# Autodesk Inventor assembly: Injector Assembly
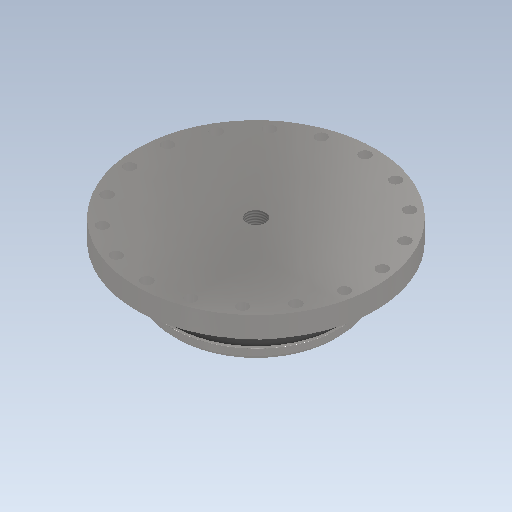
[picture p0: Inventor's stored thumbnail of the model, 512x512]
Saved by Autodesk Inventor 2021 (Build 250183000, 183)
## iProperties
Created: 2021-10-02
Part Number: Injector Assembly
Document SubType Name: Assembly
Designer: robin
Mass: 2402.63 g
Surface Area: 1092.65 cm^2
Volume: 384.578 cm^3
Density: 6.24745 g/cm^3
Author: robin
## Documents named in this file (9)
- C:\Users\alexc\OneDrive\Desktop\ATLAS\ODSY-0003 (COMBUSTION CHAMBER)\ODSY-0003-200 (INJECTOR)\ODSY-0003-200.iam
- C:\Users\alexc\OneDrive\Desktop\ATLAS\ODSY-0003 (COMBUSTION CHAMBER)\ODSY-0003-200 (INJECTOR)\ODSY-0003-201.ipt
- C:\Users\alexc\OneDrive\Desktop\ATLAS\ODSY-0003 (COMBUSTION CHAMBER)\ODSY-0003-200 (INJECTOR)\ODSY-0003-203.ipt
- C:\Users\alexc\OneDrive\Desktop\ATLAS\ODSY-0003 (COMBUSTION CHAMBER)\ODSY-0003-200 (INJECTOR)\ODSY-0003-202.ipt
- C:\Users\alexc\OneDrive\Desktop\ATLAS\ODSY-0003 (COMBUSTION CHAMBER)\ODSY-0003-200 (INJECTOR)\92185A336.ipt
- C:\Users\alexc\OneDrive\Desktop\ATLAS\ODSY-0003 (COMBUSTION CHAMBER)\ODSY-0003-200 (INJECTOR)\90945A760.ipt
- C:\Users\alexc\OneDrive\Desktop\ATLAS\ODSY-0003 (COMBUSTION CHAMBER)\ODSY-0003-200 (INJECTOR)\2-023.ipt
- C:\Users\alexc\OneDrive\Desktop\ATLAS\ODSY-0003 (COMBUSTION CHAMBER)\ODSY-0003-200 (INJECTOR)\2-030.ipt
- C:\Users\alexc\OneDrive\Desktop\ATLAS\ODSY-0003 (COMBUSTION CHAMBER)\ODSY-0003-200 (INJECTOR)\2-240.ipt
## Components (19 placed, 8 different names)
1. ODSY-0003-201:1 — Flush:1, Flush:2, Flush:3, Mate:7, Mate:8, Mate:9, Mate:10, Mate:41, Mate:42, Flush:4, Flush:5
2. ODSY-0003-203:1 — Mate:7, Mate:11, Mate:12, Mate:13, Mate:14, Mate:15, Mate:16, Mate:17, Mate:18, Mate:21, Mate:24, Mate:27, Mate:30, Mate:33, Mate:36
3. ODSY-0003-202:1 — Mate:8, Mate:9, Mate:10, Mate:11, Mate:12, Mate:37, Mate:38, Tangent:1, Tangent:2
4. 92185A336:1 — Mate:13, Mate:19, Mate:20
5. 92185A336:2 — Mate:14, Mate:25, Mate:26
6. 92185A336:3 — Mate:15, Mate:28, Mate:29
7. 92185A336:4 — Mate:16, Mate:31, Mate:32
8. 92185A336:5 — Mate:17, Mate:34, Mate:35
9. 92185A336:6 — Mate:18, Mate:22, Mate:23
10. 90945A760:1 — Mate:19, Mate:20, Mate:21
11. 90945A760:2 — Mate:25, Mate:26, Mate:27
12. 90945A760:3 — Mate:22, Mate:23, Mate:24
13. 90945A760:4 — Mate:34, Mate:35, Mate:36
14. 90945A760:5 — Mate:31, Mate:32, Mate:33
15. 90945A760:6 — Mate:28, Mate:29, Mate:30
16. 2-023:1 — Mate:37, Mate:39, Tangent:2
17. 2-030:1 — Mate:38, Mate:40, Tangent:1
18. 2-240:1 — Mate:42, Mate:43, Flush:5
19. 2-240:2 — Mate:41, Mate:44, Flush:4
## Relationships (45: Mate 38, Flush 5, Tangent 2)
- Flush:1: ODSY-0003-201:1
- Flush:2: ODSY-0003-201:1
- Flush:3: ODSY-0003-201:1
- Mate:7: ODSY-0003-201:1 ↔ ODSY-0003-203:1
- Mate:8: ODSY-0003-201:1 ↔ ODSY-0003-202:1
- Mate:9: ODSY-0003-201:1 ↔ ODSY-0003-202:1
- Mate:10: ODSY-0003-201:1 ↔ ODSY-0003-202:1
- Mate:11: ODSY-0003-203:1 ↔ ODSY-0003-202:1
- Mate:12: ODSY-0003-203:1 ↔ ODSY-0003-202:1
- Mate:13: ODSY-0003-203:1 ↔ 92185A336:1
- Mate:14: ODSY-0003-203:1 ↔ 92185A336:2
- Mate:15: ODSY-0003-203:1 ↔ 92185A336:3
- Mate:16: ODSY-0003-203:1 ↔ 92185A336:4
- Mate:17: ODSY-0003-203:1 ↔ 92185A336:5
- Mate:18: ODSY-0003-203:1 ↔ 92185A336:6
- Mate:19: 92185A336:1 ↔ 90945A760:1
- Mate:20: 92185A336:1 ↔ 90945A760:1
- Mate:21: ODSY-0003-203:1 ↔ 90945A760:1
- Mate:22: 92185A336:6 ↔ 90945A760:3
- Mate:23: 92185A336:6 ↔ 90945A760:3
- Mate:24: ODSY-0003-203:1 ↔ 90945A760:3
- Mate:25: 92185A336:2 ↔ 90945A760:2
- Mate:26: 92185A336:2 ↔ 90945A760:2
- Mate:27: ODSY-0003-203:1 ↔ 90945A760:2
- Mate:28: 92185A336:3 ↔ 90945A760:6
- Mate:29: 92185A336:3 ↔ 90945A760:6
- Mate:30: ODSY-0003-203:1 ↔ 90945A760:6
- Mate:31: 92185A336:4 ↔ 90945A760:5
- Mate:32: 92185A336:4 ↔ 90945A760:5
- Mate:33: ODSY-0003-203:1 ↔ 90945A760:5
- Mate:34: 92185A336:5 ↔ 90945A760:4
- Mate:35: 92185A336:5 ↔ 90945A760:4
- Mate:36: ODSY-0003-203:1 ↔ 90945A760:4
- Mate:37: ODSY-0003-202:1 ↔ 2-023:1
- Mate:38: ODSY-0003-202:1 ↔ 2-030:1
- Mate:39: 2-023:1
- Mate:40: 2-030:1
- Mate:41: ODSY-0003-201:1 ↔ 2-240:2
- Mate:42: ODSY-0003-201:1 ↔ 2-240:1
- Mate:43: 2-240:1
- Mate:44: 2-240:2
- Flush:4: ODSY-0003-201:1 ↔ 2-240:2
- Flush:5: ODSY-0003-201:1 ↔ 2-240:1
- Tangent:1: ODSY-0003-202:1 ↔ 2-030:1
- Tangent:2: ODSY-0003-202:1 ↔ 2-023:1
